# Autodesk Inventor assembly: Dash-V3
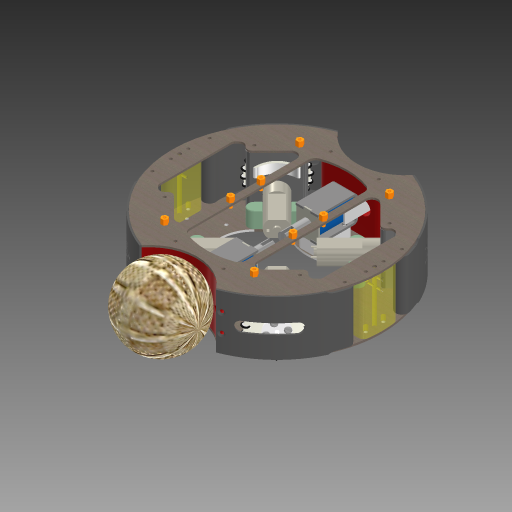
[picture p0: Inventor's stored thumbnail of the model, 512x512]
Saved by Autodesk Inventor 2023 (Build 270158000, 158)
## iProperties
Created: 2025-04-11
Part Number: Dash-V3
Document SubType Name: Assembly
Designer: Ivan
Author: Ivan
## Documents named in this file (17)
- C:\!projects\dash_localDirectory\DASH_\Dash-V1\Dash-V3.iam
- C:\!projects\dash_localDirectory\DASH_\Dash-V1\floor_v3.ipt
- C:\!projects\dash_localDirectory\DASH_\Dash-V1\Solenoid\Подставка под солноид.ipt
- C:\!projects\dash_localDirectory\DASH_\Dash-V1\Solenoid\Solenoid.iam
- C:\Users\Ivan\Documents\Inventor\Content Center Files\R2023\ru-RU\ANSI B18.2.4.2M\ANSI B18.2.4.2M - M5x0,8 - 8.ipt
- C:\!projects\dash_localDirectory\DASH_\Dash-V1\Solenoid\kicker1.1.ipt
- C:\!projects\dash_localDirectory\DASH_\Dash-V1\catch_v2.ipt
- C:\!projects\dash_localDirectory\DASH_\Dash-V1\motor_mount\motor_mount_edge_v2.ipt
- C:\!projects\dash_localDirectory\DASH_\Dash-V1\motor_mount\motor_mount_part2_v2.ipt
- C:\!projects\dash_localDirectory\DASH_\Dash-V1\motor20.ipt
- C:\!projects\dash_localDirectory\DASH_\Dash-V1\protect_v2.2.ipt
- C:\!projects\dash_localDirectory\DASH_\Dash-V1\protect_v2.2_dash.ipt
- C:\!projects\dash_localDirectory\DASH_\Dash-V1\wheel\Wheel.iam
- C:\!projects\dash_localDirectory\DASH_\Dash-V1\contour_v3.ipt
- C:\!projects\dash_localDirectory\DASH_\Dash-V1\ball.ipt
- C:\!projects\dash_localDirectory\DASH_\Dash-V1\крепление ручки.ipt
- C:\!projects\dash_localDirectory\DASH_\Dash-V1\step\m3_bolt\Spacer Bolts_m3_bn_L5.ipt
## Components (43 placed, 15 different names)
1. floor_v3:1 — Совмещение:1, Совмещение:2, Вставка:1, Вставка:2, Угол:5, Угол:6, Вставка:9, Вставка:10, Вставка:11, Вставка:12, Вставка:13, Вставка:14, Вставка:15, Вставка:16, Вставка:17, Вставка:18, Вставка:23, Вставка:24, Вставка:25, Вставка:26, Заподлицо:2, Заподлицо:3, Вставка:33, Вставка:34
2. Подставка под солноид:1 — Совмещение:1, Вставка:1, Угол:1, Совмещение:3, Вставка:3, Угол:4
3. Подставка под солноид:2 — Совмещение:2, Вставка:2, Угол:2, Совмещение:4, Вставка:4, Угол:3
4. Solenoid:1 [sub-assembly] — Совмещение:3, Вставка:3, Угол:4, Вставка:7, Угол:8
5. Solenoid:2 [sub-assembly] — Совмещение:4, Вставка:4, Угол:3, Вставка:8, Угол:7
6. ANSI B18.2.4.2M M5x0,8:1 — Вставка:6
7. ANSI B18.2.4.2M M5x0,8:2 — Вставка:5
8. kicker1.1:1 — Вставка:6, Вставка:7, Угол:6
9. kicker1.1:2 — Вставка:5, Вставка:8, Угол:5
10. catch_v2:1 — Вставка:10, Угол:7, Касательность:1, Касательность:3, Вставка:31
11. catch_v2:2 — Вставка:9, Угол:8, Угол:9, Касательность:2, Касательность:4, Вставка:32
12. motor_mount_edge_v2:1 — Вставка:15, Угол:9, Угол:10, Угол:11, Вставка:20, Вставка:28
13. motor_mount_part2_v2:1 — Вставка:11, Угол:15, Угол:16, Угол:19
14. motor_mount_edge_v2:2 — Вставка:16, Угол:10, Угол:12, Угол:13, Вставка:19, Вставка:27
15. motor_mount_part2_v2:2 — Вставка:13, Угол:16, Угол:17
16. motor_mount_edge_v2:3 — Вставка:17, Угол:11, Вставка:22, Вставка:30
17. motor_mount_part2_v2:3 — Вставка:12, Угол:13, Угол:14, Угол:15, Угол:20
18. motor_mount_edge_v2:4 — Вставка:18, Угол:12, Вставка:21, Вставка:29
19. motor_mount_part2_v2:4 — Вставка:14, Угол:14, Угол:18
20. motor20:1 — Вставка:19, Угол:20, Угол:21
21. motor20:2 — Вставка:20, Угол:19, Угол:22
22. motor20:3 — Вставка:21, Угол:18, Угол:23
23. motor20:4 — Вставка:22, Угол:17, Угол:24
24. protect_v2:1 — Вставка:24, Касательность:4
25. protect_v2:2 — Вставка:23, Касательность:1
26. protect_v2:3 — Вставка:26, Касательность:2
27. protect_v2:4 — Вставка:25, Касательность:3
28. Wheel:1 [sub-assembly] — Вставка:27, Угол:21
29. Wheel:2 [sub-assembly] — Вставка:28, Угол:22
30. Wheel:3 [sub-assembly] — Вставка:29, Угол:23
31. Wheel:4 [sub-assembly] — Вставка:30, Угол:24
32. contour:1 — Вставка:31, Вставка:32, Совмещение:5, Вставка:35, Вставка:36, Вставка:37, Вставка:38, Вставка:39, Вставка:40, Вставка:41, Вставка:42
33. ball:1 — Касательность:5
34. крепление ручки:1 — Заподлицо:2, Заподлицо:3
35. крепление ручки:2 — Вставка:33, Вставка:34
36. Spacer Bolts_m3_bn_L5:1 — Вставка:42
37. Spacer Bolts_m3_bn_L5:2 — Вставка:41
38. Spacer Bolts_m3_bn_L5:3 — Вставка:40
39. Spacer Bolts_m3_bn_L5:4 — Вставка:38
40. Spacer Bolts_m3_bn_L5:5 — Вставка:39
41. Spacer Bolts_m3_bn_L5:6 — Вставка:37
42. Spacer Bolts_m3_bn_L5:7 — Вставка:35
43. Spacer Bolts_m3_bn_L5:8 — Вставка:36
## Relationships (79: Insert 42, Angle 24, Mate 5, Tangent 5, Flush 3)
- Совмещение:1 [Mate]: floor_v3:1 ↔ Подставка под солноид:1
- Совмещение:2 [Mate]: floor_v3:1 ↔ Подставка под солноид:2
- Вставка:1 [Insert]: floor_v3:1 ↔ Подставка под солноид:1
- Вставка:2 [Insert]: floor_v3:1 ↔ Подставка под солноид:2
- Угол:1 [Angle] (0 deg): Подставка под солноид:1
- Угол:2 [Angle] (0 deg): Подставка под солноид:2
- Совмещение:3 [Mate]: Подставка под солноид:1 ↔ Solenoid:1
- Совмещение:4 [Mate]: Подставка под солноид:2 ↔ Solenoid:2
- Вставка:3 [Insert]: Подставка под солноид:1 ↔ Solenoid:1
- Вставка:4 [Insert]: Подставка под солноид:2 ↔ Solenoid:2
- Угол:3 [Angle] (0 deg): Подставка под солноид:2 ↔ Solenoid:2
- Угол:4 [Angle] (0 deg): Подставка под солноид:1 ↔ Solenoid:1
- Вставка:5 [Insert]: ANSI B18.2.4.2M M5x0,8:2 ↔ kicker1.1:2
- Вставка:6 [Insert]: ANSI B18.2.4.2M M5x0,8:1 ↔ kicker1.1:1
- Вставка:7 [Insert]: Solenoid:1 ↔ kicker1.1:1
- Вставка:8 [Insert]: Solenoid:2 ↔ kicker1.1:2
- Угол:5 [Angle] (0 deg): floor_v3:1 ↔ kicker1.1:2
- Угол:6 [Angle] (0 deg): floor_v3:1 ↔ kicker1.1:1
- Вставка:9 [Insert]: floor_v3:1 ↔ catch_v2:2
- Вставка:10 [Insert]: floor_v3:1 ↔ catch_v2:1
- Угол:7 [Angle] (180 deg): Solenoid:2 ↔ catch_v2:1
- Угол:8 [Angle] (180 deg): Solenoid:1 ↔ catch_v2:2
- Вставка:11 [Insert]: floor_v3:1 ↔ motor_mount_part2_v2:1
- Вставка:12 [Insert]: floor_v3:1 ↔ motor_mount_part2_v2:3
- Вставка:13 [Insert]: floor_v3:1 ↔ motor_mount_part2_v2:2
- Вставка:14 [Insert]: floor_v3:1 ↔ motor_mount_part2_v2:4
- Вставка:15 [Insert]: floor_v3:1 ↔ motor_mount_edge_v2:1
- Вставка:16 [Insert]: floor_v3:1 ↔ motor_mount_edge_v2:2
- Вставка:17 [Insert]: floor_v3:1 ↔ motor_mount_edge_v2:3
- Вставка:18 [Insert]: floor_v3:1 ↔ motor_mount_edge_v2:4
- Угол:9 [Angle] (135 deg): catch_v2:2 ↔ motor_mount_edge_v2:1
- Угол:10 [Angle] (270 deg): motor_mount_edge_v2:1 ↔ motor_mount_edge_v2:2
- Угол:11 [Angle] (180 deg): motor_mount_edge_v2:1 ↔ motor_mount_edge_v2:3
- Угол:12 [Angle] (180 deg): motor_mount_edge_v2:2 ↔ motor_mount_edge_v2:4
- Угол:13 [Angle] (180 deg): motor_mount_edge_v2:2 ↔ motor_mount_part2_v2:3
- Угол:14 [Angle] (180 deg): motor_mount_part2_v2:3 ↔ motor_mount_part2_v2:4
- Угол:15 [Angle] (90 deg): motor_mount_part2_v2:1 ↔ motor_mount_part2_v2:3
- Угол:16 [Angle] (0 deg): motor_mount_part2_v2:1 ↔ motor_mount_part2_v2:2
- Вставка:19 [Insert]: motor_mount_edge_v2:2 ↔ motor20:1
- Вставка:20 [Insert]: motor_mount_edge_v2:1 ↔ motor20:2
- Вставка:21 [Insert]: motor_mount_edge_v2:4 ↔ motor20:3
- Вставка:22 [Insert]: motor_mount_edge_v2:3 ↔ motor20:4
- Угол:17 [Angle] (0 deg): motor_mount_part2_v2:2 ↔ motor20:4
- Угол:18 [Angle] (0 deg): motor_mount_part2_v2:4 ↔ motor20:3
- Угол:19 [Angle] (0 deg): motor_mount_part2_v2:1 ↔ motor20:2
- Угол:20 [Angle] (0 deg): motor_mount_part2_v2:3 ↔ motor20:1
- Вставка:23 [Insert]: floor_v3:1 ↔ protect_v2:2
- Вставка:24 [Insert]: floor_v3:1 ↔ protect_v2:1
- Вставка:25 [Insert]: floor_v3:1 ↔ protect_v2:4
- Вставка:26 [Insert]: floor_v3:1 ↔ protect_v2:3
- Касательность:1 [Tangent]: catch_v2:1 ↔ protect_v2:2
- Касательность:2 [Tangent]: catch_v2:2 ↔ protect_v2:3
- Касательность:3 [Tangent]: catch_v2:1 ↔ protect_v2:4
- Касательность:4 [Tangent]: catch_v2:2 ↔ protect_v2:1
- Вставка:27 [Insert]: motor_mount_edge_v2:2 ↔ Wheel:1
- Вставка:28 [Insert]: motor_mount_edge_v2:1 ↔ Wheel:2
- Вставка:29 [Insert]: motor_mount_edge_v2:4 ↔ Wheel:3
- Вставка:30 [Insert]: motor_mount_edge_v2:3 ↔ Wheel:4
- Угол:21 [Angle] (0 deg): motor20:1 ↔ Wheel:1
- Угол:22 [Angle] (0 deg): motor20:2 ↔ Wheel:2
- Угол:23 [Angle] (0 deg): motor20:3 ↔ Wheel:3
- Угол:24 [Angle] (0 deg): motor20:4 ↔ Wheel:4
- Вставка:31 [Insert]: catch_v2:1 ↔ contour:1
- Вставка:32 [Insert]: catch_v2:2 ↔ contour:1
- Заподлицо:1 [Flush] (-3 mm)
- Касательность:5 [Tangent]: ball:1
- Совмещение:5 [Mate]: contour:1
- Заподлицо:2 [Flush]: floor_v3:1 ↔ крепление ручки:1
- Заподлицо:3 [Flush]: floor_v3:1 ↔ крепление ручки:1
- Вставка:33 [Insert]: floor_v3:1 ↔ крепление ручки:2
- Вставка:34 [Insert]: floor_v3:1 ↔ крепление ручки:2
- Вставка:35 [Insert]: contour:1 ↔ Spacer Bolts_m3_bn_L5:7
- Вставка:36 [Insert]: contour:1 ↔ Spacer Bolts_m3_bn_L5:8
- Вставка:37 [Insert]: contour:1 ↔ Spacer Bolts_m3_bn_L5:6
- Вставка:38 [Insert]: contour:1 ↔ Spacer Bolts_m3_bn_L5:4
- Вставка:39 [Insert]: contour:1 ↔ Spacer Bolts_m3_bn_L5:5
- Вставка:40 [Insert]: contour:1 ↔ Spacer Bolts_m3_bn_L5:3
- Вставка:41 [Insert]: contour:1 ↔ Spacer Bolts_m3_bn_L5:2
- Вставка:42 [Insert]: contour:1 ↔ Spacer Bolts_m3_bn_L5:1
